# Autodesk Inventor assembly: assemblage_base_amovible
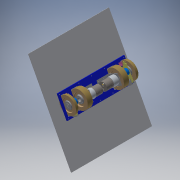
[picture p0: Inventor's stored thumbnail of the model, 180x180]
Saved by Autodesk Inventor 2017 (Build 210142000, 142)
## iProperties
Created: 2017-04-12
Part Number: assemblage_base_amovible
Document SubType Name: Assembly
Designer: franc
Author: franc
## Documents named in this file (14)
- C:\Users\franc\Desktop\EsialRobotik\Mecanique\base roulante\assemblage_base_amovible.iam
- C:\Users\franc\Desktop\EsialRobotik\Mecanique\base roulante\base_roulante.ipt
- C:\Users\franc\Desktop\EsialRobotik\Mecanique\base roulante\support_moteur.ipt
- C:\Users\franc\Desktop\EsialRobotik\Mecanique\base roulante\37d-gearmotor-19-30.ipt
- C:\Users\franc\Desktop\EsialRobotik\Mecanique\base roulante\moyeu_serrage_conique.ipt
- C:\Users\franc\Desktop\EsialRobotik\Mecanique\base roulante\Colson_Wheel_3in_x_7_8in.ipt
- C:\Users\franc\Desktop\EsialRobotik\Mecanique\base roulante\palier_roulement_bras.ipt
- C:\Users\franc\Desktop\EsialRobotik\Mecanique\base roulante\bras_amortisseur.ipt
- C:\Users\franc\Desktop\EsialRobotik\Mecanique\base roulante\Codeur.ipt
- C:\Users\franc\Desktop\EsialRobotik\Mecanique\base roulante\T40_hub_40mm_1screw.ipt
- C:\Users\franc\Desktop\EsialRobotik\Mecanique\base roulante\T40_Wheel_2_875in_x_0_5in.ipt
- C:\Users\franc\Desktop\EsialRobotik\Mecanique\base roulante\sol.ipt
- C:\Users\franc\Desktop\EsialRobotik\Mecanique\base roulante\crochet.ipt
- C:\Users\franc\Desktop\EsialRobotik\Mecanique\base roulante\crochet2.ipt
## Components (22 placed, 13 different names)
1. base_roulante:1 — Mate:19, Mate:20, Mate:21, Mate:22, Mate:23, Mate:24, Angle:1, Flush:3, Flush:4, Mate:49, Mate:50, Mate:51, Mate:52, Mate:53, Mate:54, Mate:59, Mate:60, Mate:61, Mate:62, Mate:63, Mate:64
2. 37d-gearmotor-19-30:1 — Mate:13, Mate:14, Mate:66, Mate:67, Mate:68
3. 37d-gearmotor-19-30:2 — Mate:15, Mate:16, Mate:56, Mate:58, Mate:69
4. moyeu_serrage_conique:1 — Mate:13, Mate:14, Mate:18, Flush:2
5. moyeu_serrage_conique:2 — Mate:15, Mate:16, Mate:17, Flush:1
6. Colson_Wheel_3in_x_7_8in:1 — Mate:17, Flush:1, Mate:70
7. Colson_Wheel_3in_x_7_8in:2 — Mate:18, Flush:2, Mate:44, Mate:71, Tangent:1
8. palier_roulement_bras:1 — Mate:19, Mate:20, Mate:21, Mate:28, Mate:29
9. palier_roulement_bras:2 — Mate:22, Mate:23, Mate:24, Mate:30, Mate:31
10. bras_amortisseur:1 — Mate:25, Mate:26, Mate:27, Mate:28, Mate:29, Mate:36
11. bras_amortisseur:2 — Mate:30, Mate:31, Mate:32, Mate:33, Mate:34, Mate:38
12. Codeur:1 — Mate:25, Mate:26, Mate:27, Mate:35
13. Codeur:2 — Mate:32, Mate:33, Mate:34, Mate:37
14. T40_hub_40mm_1screw:1 — Mate:35, Mate:36, Mate:39, Mate:40
15. T40_hub_40mm_1screw:2 — Mate:37, Mate:38, Mate:41, Mate:42
16. T40_Wheel_2_875in_x_0_5in:1 — Mate:39, Mate:40, Mate:70
17. T40_Wheel_2_875in_x_0_5in:2 — Mate:41, Mate:42, Mate:71
18. sol:1 — Mate:44, Angle:1, Flush:3, Flush:4, Tangent:1
19. crochet:1 — Mate:49, Mate:50, Mate:51
20. crochet2:1 — Mate:52, Mate:53, Mate:54
21. support_moteur:1 — Mate:56, Mate:58, Mate:59, Mate:60, Mate:61, Mate:69
22. support_moteur:2 — Mate:62, Mate:63, Mate:64, Mate:66, Mate:67, Mate:68
## Relationships (57: Mate 51, Flush 4, Angle 1, Tangent 1)
- Mate:13: 37d-gearmotor-19-30:1 ↔ moyeu_serrage_conique:1
- Mate:14: 37d-gearmotor-19-30:1 ↔ moyeu_serrage_conique:1
- Mate:15: 37d-gearmotor-19-30:2 ↔ moyeu_serrage_conique:2
- Mate:16: 37d-gearmotor-19-30:2 ↔ moyeu_serrage_conique:2
- Mate:17: moyeu_serrage_conique:2 ↔ Colson_Wheel_3in_x_7_8in:1
- Flush:1: moyeu_serrage_conique:2 ↔ Colson_Wheel_3in_x_7_8in:1
- Mate:18: moyeu_serrage_conique:1 ↔ Colson_Wheel_3in_x_7_8in:2
- Flush:2: moyeu_serrage_conique:1 ↔ Colson_Wheel_3in_x_7_8in:2
- Mate:19: base_roulante:1 ↔ palier_roulement_bras:1
- Mate:20: base_roulante:1 ↔ palier_roulement_bras:1
- Mate:21: base_roulante:1 ↔ palier_roulement_bras:1
- Mate:22: base_roulante:1 ↔ palier_roulement_bras:2
- Mate:23: base_roulante:1 ↔ palier_roulement_bras:2
- Mate:24: base_roulante:1 ↔ palier_roulement_bras:2
- Mate:25: bras_amortisseur:1 ↔ Codeur:1
- Mate:26: bras_amortisseur:1 ↔ Codeur:1
- Mate:27: bras_amortisseur:1 ↔ Codeur:1
- Mate:28: palier_roulement_bras:1 ↔ bras_amortisseur:1
- Mate:29: palier_roulement_bras:1 ↔ bras_amortisseur:1
- Mate:30: palier_roulement_bras:2 ↔ bras_amortisseur:2
- Mate:31: palier_roulement_bras:2 ↔ bras_amortisseur:2
- Mate:32: bras_amortisseur:2 ↔ Codeur:2
- Mate:33: bras_amortisseur:2 ↔ Codeur:2
- Mate:34: bras_amortisseur:2 ↔ Codeur:2
- Mate:35: Codeur:1 ↔ T40_hub_40mm_1screw:1
- Mate:36 (1 mm): bras_amortisseur:1 ↔ T40_hub_40mm_1screw:1
- Mate:37: Codeur:2 ↔ T40_hub_40mm_1screw:2
- Mate:38 (1 mm): bras_amortisseur:2 ↔ T40_hub_40mm_1screw:2
- Mate:39: T40_hub_40mm_1screw:1 ↔ T40_Wheel_2_875in_x_0_5in:1
- Mate:40: T40_hub_40mm_1screw:1 ↔ T40_Wheel_2_875in_x_0_5in:1
- Mate:41: T40_hub_40mm_1screw:2 ↔ T40_Wheel_2_875in_x_0_5in:2
- Mate:42: T40_hub_40mm_1screw:2 ↔ T40_Wheel_2_875in_x_0_5in:2
- Mate:44: Colson_Wheel_3in_x_7_8in:2 ↔ sol:1
- Angle:1 (0 deg): base_roulante:1 ↔ sol:1
- Flush:3 (150 mm): base_roulante:1 ↔ sol:1
- Flush:4 (-25 mm): base_roulante:1 ↔ sol:1
- Mate:49: base_roulante:1 ↔ crochet:1
- Mate:50: base_roulante:1 ↔ crochet:1
- Mate:51: base_roulante:1 ↔ crochet:1
- Mate:52: base_roulante:1 ↔ crochet2:1
- Mate:53: base_roulante:1 ↔ crochet2:1
- Mate:54: base_roulante:1 ↔ crochet2:1
- Mate:56: 37d-gearmotor-19-30:2 ↔ support_moteur:1
- Mate:58: 37d-gearmotor-19-30:2 ↔ support_moteur:1
- Mate:59: base_roulante:1 ↔ support_moteur:1
- Mate:60: base_roulante:1 ↔ support_moteur:1
- Mate:61: base_roulante:1 ↔ support_moteur:1
- Mate:62: base_roulante:1 ↔ support_moteur:2
- Mate:63: base_roulante:1 ↔ support_moteur:2
- Mate:64: base_roulante:1 ↔ support_moteur:2
- Mate:66: 37d-gearmotor-19-30:1 ↔ support_moteur:2
- Mate:67: 37d-gearmotor-19-30:1 ↔ support_moteur:2
- Mate:68: 37d-gearmotor-19-30:1 ↔ support_moteur:2
- Mate:69: 37d-gearmotor-19-30:2 ↔ support_moteur:1
- Mate:70: Colson_Wheel_3in_x_7_8in:1 ↔ T40_Wheel_2_875in_x_0_5in:1
- Mate:71: Colson_Wheel_3in_x_7_8in:2 ↔ T40_Wheel_2_875in_x_0_5in:2
- Tangent:1: Colson_Wheel_3in_x_7_8in:2 ↔ sol:1
